# Autodesk Inventor assembly: Carro
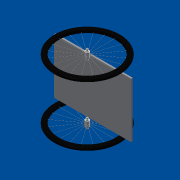
[picture p0: Inventor's stored thumbnail of the model, 180x180]
Saved by Autodesk Inventor 2016 (Build 200138000, 138)
## iProperties
Created: 2017-05-14
Part Number: Carro
Document SubType Name: Assembly
Designer: Gian
Author: Gian
## Documents named in this file (3)
- C:\Users\Gian\Desktop\Pedalazo\002_Diseño\Version_001\Carro.iam
- C:\Users\Gian\Desktop\Pedalazo\002_Diseño\Version_001\Rueda.ipt
- C:\Users\Gian\Desktop\Pedalazo\002_Diseño\Version_001\Base.ipt
## Components (3 placed, 2 different names)
1. Rueda:1 — Cylindrical:1
2. Rueda:2 — Cylindrical:1
3. Base:1
## Relationships (1: CylindricalJoint 1)
- Cylindrical:1: Rueda:1 ↔ Rueda:2
